# Autodesk Inventor assembly: supportForWinch
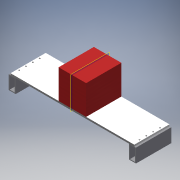
[picture p0: Inventor's stored thumbnail of the model, 180x180]
Saved by Autodesk Inventor 2018.2 (Build 222227000, 227)
## iProperties
Created: 2018-01-10
Part Number: supportForWinch
Document SubType Name: Assembly
Designer: steele
Author: steele
## Documents named in this file (5)
- D:\snobotics\CAD-Development\robSteele\2018-FRC\supportForWinch.iam
- D:\snobotics\CAD-Development\robSteele\2018-FRC\AluminumPlateForWinch.ipt
- D:\snobotics\CAD-Development\robSteele\2018-FRC\WinchVolume.ipt
- D:\snobotics\CAD-Development\robSteele\2018-FRC\SupportForWinchSupport.ipt
- D:\snobotics\CAD-Development\robSteele\2018-FRC\SupportForWinchSupport_MIR1.ipt
## Components (4 placed, 4 different names)
1. AluminumPlateForWinch:1 — Mate:6, Flush:3, Mate:7, Flush:4, Flush:5
2. WinchVolume:1 — Mate:6, Flush:3
3. SupportForWinchSupport:1 — Mate:7, Flush:4, Flush:5
4. SupportForWinchSupport_MIR1:1
## Relationships (5: Flush 3, Mate 2)
- Mate:6: AluminumPlateForWinch:1 ↔ WinchVolume:1
- Flush:3: AluminumPlateForWinch:1 ↔ WinchVolume:1
- Mate:7: AluminumPlateForWinch:1 ↔ SupportForWinchSupport:1
- Flush:4 (-6.35 mm): AluminumPlateForWinch:1 ↔ SupportForWinchSupport:1
- Flush:5: AluminumPlateForWinch:1 ↔ SupportForWinchSupport:1
